# Autodesk Inventor assembly: BC-100001-Sup
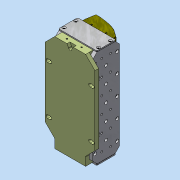
[picture p0: Inventor's stored thumbnail of the model, 180x180]
Saved by Autodesk Inventor 2016 (Build 200138000, 138)
## iProperties
Created: 2015-09-23
Part Number: BC-100001-Sup
Document SubType Name: Assembly
Designer: Reinaldo.Basílio
Mass: 35341.7 g
Surface Area: 4837.15 cm^2
Volume: 4562.02 cm^3
Density: 7.74696 g/cm^3
Author: Reinaldo.Basílio
## Documents named in this file (6)
- D:\ARQ\Basilio\LNLS-2\Anel\Dipolos\BC-3T\Dipolo 3T e 1T\Prototipo 1\Projeto Mecanico\BC-100001-Sup.iam
- D:\ARQ\Basilio\LNLS-2\Anel\Dipolos\BC-3T\Dipolo 3T e 1T\Prototipo 1\Projeto Mecanico\BC-100002.iam
- D:\ARQ\Basilio\LNLS-2\Anel\Dipolos\BC-3T\Dipolo 3T e 1T\Prototipo 1\Projeto Mecanico\BC-10003-A.ipt
- D:\ARQ\Basilio\LNLS-2\Anel\Dipolos\BC-3T\Dipolo 3T e 1T\Prototipo 1\Projeto Mecanico\BC-10004.ipt
- D:\ARQ\Basilio\LNLS-2\Anel\Dipolos\BC-3T\Dipolo 3T e 1T\Prototipo 1\Projeto Mecanico\BC-10017.ipt
- D:\ARQ\Basilio\LNLS-2\Anel\Dipolos\BC-3T\Dipolo 3T e 1T\Prototipo 1\Projeto Mecanico\BC-10024.ipt
## Components (7 placed, 5 different names)
1. BC-10003-A:1 — Flush:10, Mate:4, Mate:5, Flush:12, Flush:13, Mate:13
2. BC-100002:1 [sub-assembly] — Flush:7, Mate:12, Mate:6, Mate:13
3. BC-10004:1 — Flush:7, Mate:12, Flush:12, Flush:13, Insert:2, Insert:3, Mate:6, Insert:9
4. BC-10017:1 — Insert:2, Insert:6, Insert:8
5. BC-10017:2 — Insert:3, Insert:5, Insert:7, Insert:9
6. BC-10024:1 — Insert:5, Insert:6
7. BC-10024:2 — Insert:7, Insert:8
## Relationships (16: Insert 7, Mate 5, Flush 4)
- Flush:7: BC-100002:1 ↔ BC-10004:1
- Flush:10: BC-10003-A:1
- Mate:4: BC-10003-A:1
- Mate:5 (-57.5 mm): BC-10003-A:1
- Mate:12: BC-100002:1 ↔ BC-10004:1
- Flush:12: BC-10003-A:1 ↔ BC-10004:1
- Flush:13: BC-10003-A:1 ↔ BC-10004:1
- Insert:2: BC-10004:1 ↔ BC-10017:1
- Insert:3: BC-10004:1 ↔ BC-10017:2
- Mate:6: BC-100002:1 ↔ BC-10004:1
- Insert:5: BC-10017:2 ↔ BC-10024:1
- Insert:6: BC-10017:1 ↔ BC-10024:1
- Insert:7: BC-10017:2 ↔ BC-10024:2
- Insert:8: BC-10017:1 ↔ BC-10024:2
- Mate:13: BC-10003-A:1 ↔ BC-100002:1
- Insert:9: BC-10004:1 ↔ BC-10017:2
